# Autodesk Inventor assembly: Assembly
(part 3 of 3)
54. Universal_board_70x90mm_31x26-prt53
55. Universal_board_70x90mm_31x26-prt54
56. Universal_board_70x90mm_31x26-prt55
57. Universal_board_70x90mm_31x26-prt56
58. Universal_board_70x90mm_31x26-prt57
59. Universal_board_70x90mm_31x26-prt58
60. Universal_board_70x90mm_31x26-prt59
61. Universal_board_70x90mm_31x26-prt60
62. Universal_board_70x90mm_31x26-prt61
63. Universal_board_70x90mm_31x26-prt62
64. Universal_board_70x90mm_31x26-prt63
65. Universal_board_70x90mm_31x26-prt64
66. Universal_board_70x90mm_31x26-prt65
67. Universal_board_70x90mm_31x26-prt66
68. Universal_board_70x90mm_31x26-prt67
69. Universal_board_70x90mm_31x26-prt68
70. Universal_board_70x90mm_31x26-prt69
71. Universal_board_70x90mm_31x26-prt70
72. Universal_board_70x90mm_31x26-prt71
73. Universal_board_70x90mm_31x26-prt72
74. Universal_board_70x90mm_31x26-prt73
75. Universal_board_70x90mm_31x26-prt74
76. Universal_board_70x90mm_31x26-prt75
77. Universal_board_70x90mm_31x26-prt76
78. Universal_board_70x90mm_31x26-prt77
79. Universal_board_70x90mm_31x26-prt78
80. Universal_board_70x90mm_31x26-prt79
81. Universal_board_70x90mm_31x26-prt80
82. Universal_board_70x90mm_31x26-prt81
83. Universal_board_70x90mm_31x26-prt82
84. Universal_board_70x90mm_31x26-prt83
85. Universal_board_70x90mm_31x26-prt84
86. Universal_board_70x90mm_31x26-prt85
87. Universal_board_70x90mm_31x26-prt86
88. Universal_board_70x90mm_31x26-prt87
89. Universal_board_70x90mm_31x26-prt88
90. Universal_board_70x90mm_31x26-prt89
91. Universal_board_70x90mm_31x26-prt90
92. Universal_board_70x90mm_31x26-prt91
93. Universal_board_70x90mm_31x26-prt92
94. Universal_board_70x90mm_31x26-prt93
95. Universal_board_70x90mm_31x26-prt94
96. Universal_board_70x90mm_31x26-prt95
97. Universal_board_70x90mm_31x26-prt96
98. Universal_board_70x90mm_31x26-prt97
99. Universal_board_70x90mm_31x26-prt98
100. Universal_board_70x90mm_31x26-prt99
101. Universal_board_70x90mm_31x26-prt100
102. Universal_board_70x90mm_31x26-prt101
103. Universal_board_70x90mm_31x26-prt102
104. Universal_board_70x90mm_31x26-prt103
105. Universal_board_70x90mm_31x26-prt104
106. Universal_board_70x90mm_31x26-prt105
107. Universal_board_70x90mm_31x26-prt106
108. Universal_board_70x90mm_31x26-prt107
109. Universal_board_70x90mm_31x26-prt108
110. Universal_board_70x90mm_31x26-prt109
111. Universal_board_70x90mm_31x26-prt110
112. Universal_board_70x90mm_31x26-prt111
113. Universal_board_70x90mm_31x26-prt112
114. Universal_board_70x90mm_31x26-prt113
115. Universal_board_70x90mm_31x26-prt114
116. Universal_board_70x90mm_31x26-prt115
117. Universal_board_70x90mm_31x26-prt116
118. Universal_board_70x90mm_31x26-prt117
119. Universal_board_70x90mm_31x26-prt118
120. Universal_board_70x90mm_31x26-prt119
121. Universal_board_70x90mm_31x26-prt120
122. Universal_board_70x90mm_31x26-prt121
123. Universal_board_70x90mm_31x26-prt122
124. Universal_board_70x90mm_31x26-prt123
125. Universal_board_70x90mm_31x26-prt124
126. Universal_board_70x90mm_31x26-prt125
127. Universal_board_70x90mm_31x26-prt126
128. Universal_board_70x90mm_31x26-prt127
129. Universal_board_70x90mm_31x26-prt128
130. Universal_board_70x90mm_31x26-prt129
131. Universal_board_70x90mm_31x26-prt130
132. Universal_board_70x90mm_31x26-prt131
133. Universal_board_70x90mm_31x26-prt132
134. Universal_board_70x90mm_31x26-prt133
135. Universal_board_70x90mm_31x26-prt134
136. Universal_board_70x90mm_31x26-prt135
137. Universal_board_70x90mm_31x26-prt136
138. Universal_board_70x90mm_31x26-prt137
139. Universal_board_70x90mm_31x26-prt138
140. Universal_board_70x90mm_31x26-prt139
141. Universal_board_70x90mm_31x26-prt140
142. Universal_board_70x90mm_31x26-prt141
143. Universal_board_70x90mm_31x26-prt142
144. Universal_board_70x90mm_31x26-prt143
145. Universal_board_70x90mm_31x26-prt144
146. Universal_board_70x90mm_31x26-prt145
147. Universal_board_70x90mm_31x26-prt146
148. Universal_board_70x90mm_31x26-prt147
149. Universal_board_70x90mm_31x26-prt148
150. Universal_board_70x90mm_31x26-prt149
151. Universal_board_70x90mm_31x26-prt150
152. Universal_board_70x90mm_31x26-prt151
153. Universal_board_70x90mm_31x26-prt152
154. Universal_board_70x90mm_31x26-prt153
155. Universal_board_70x90mm_31x26-prt154
156. Universal_board_70x90mm_31x26-prt155
157. Universal_board_70x90mm_31x26-prt156
158. Universal_board_70x90mm_31x26-prt157
159. Universal_board_70x90mm_31x26-prt158
160. Universal_board_70x90mm_31x26-prt159
161. Universal_board_70x90mm_31x26-prt160
162. Universal_board_70x90mm_31x26-prt161
163. Universal_board_70x90mm_31x26-prt162
164. Universal_board_70x90mm_31x26-prt163
165. Universal_board_70x90mm_31x26-prt164
166. Universal_board_70x90mm_31x26-prt165
167. Universal_board_70x90mm_31x26-prt166
168. Universal_board_70x90mm_31x26-prt167
169. Universal_board_70x90mm_31x26-prt168
170. Universal_board_70x90mm_31x26-prt169
171. Universal_board_70x90mm_31x26-prt170
172. Universal_board_70x90mm_31x26-prt171
173. Universal_board_70x90mm_31x26-prt172
174. Universal_board_70x90mm_31x26-prt173
175. Universal_board_70x90mm_31x26-prt174
176. Universal_board_70x90mm_31x26-prt175
177. Universal_board_70x90mm_31x26-prt176
178. Universal_board_70x90mm_31x26-prt177
179. Universal_board_70x90mm_31x26-prt178
180. Universal_board_70x90mm_31x26-prt179
181. Universal_board_70x90mm_31x26-prt180
182. Universal_board_70x90mm_31x26-prt181
183. Universal_board_70x90mm_31x26-prt182
184. Universal_board_70x90mm_31x26-prt183
185. Universal_board_70x90mm_31x26-prt184
186. Universal_board_70x90mm_31x26-prt185
187. Universal_board_70x90mm_31x26-prt186
188. Universal_board_70x90mm_31x26-prt187
189. Universal_board_70x90mm_31x26-prt188
190. Universal_board_70x90mm_31x26-prt189
191. Universal_board_70x90mm_31x26-prt190
192. Universal_board_70x90mm_31x26-prt191
193. Universal_board_70x90mm_31x26-prt192
194. Universal_board_70x90mm_31x26-prt193
195. Universal_board_70x90mm_31x26-prt194
196. Universal_board_70x90mm_31x26-prt195
197. Universal_board_70x90mm_31x26-prt196
198. Universal_board_70x90mm_31x26-prt197
199. Universal_board_70x90mm_31x26-prt198
200. Universal_board_70x90mm_31x26-prt199
201. Universal_board_70x90mm_31x26-prt200
202. Universal_board_70x90mm_31x26-prt201
203. Universal_board_70x90mm_31x26-prt202
204. Universal_board_70x90mm_31x26-prt203
205. Universal_board_70x90mm_31x26-prt204
206. Universal_board_70x90mm_31x26-prt205
207. Universal_board_70x90mm_31x26-prt206
208. Universal_board_70x90mm_31x26-prt207
209. Universal_board_70x90mm_31x26-prt208
210. Universal_board_70x90mm_31x26-prt209
211. Universal_board_70x90mm_31x26-prt210
212. Universal_board_70x90mm_31x26-prt211
213. Universal_board_70x90mm_31x26-prt212
214. Universal_board_70x90mm_31x26-prt213
215. Universal_board_70x90mm_31x26-prt214
216. Universal_board_70x90mm_31x26-prt215
217. Universal_board_70x90mm_31x26-prt216
218. Universal_board_70x90mm_31x26-prt217
219. Universal_board_70x90mm_31x26-prt218
220. Universal_board_70x90mm_31x26-prt219
221. Universal_board_70x90mm_31x26-prt220
222. Universal_board_70x90mm_31x26-prt221
223. Universal_board_70x90mm_31x26-prt222
224. Universal_board_70x90mm_31x26-prt223
225. Universal_board_70x90mm_31x26-prt224
226. Universal_board_70x90mm_31x26-prt225
227. Universal_board_70x90mm_31x26-prt226
228. Universal_board_70x90mm_31x26-prt227
229. Universal_board_70x90mm_31x26-prt228
230. Universal_board_70x90mm_31x26-prt229
231. Universal_board_70x90mm_31x26-prt230
232. Universal_board_70x90mm_31x26-prt231
233. Universal_board_70x90mm_31x26-prt232
234. Universal_board_70x90mm_31x26-prt233
235. Universal_board_70x90mm_31x26-prt234
236. Universal_board_70x90mm_31x26-prt235
237. Universal_board_70x90mm_31x26-prt236
238. Universal_board_70x90mm_31x26-prt237
239. Universal_board_70x90mm_31x26-prt238
240. Universal_board_70x90mm_31x26-prt239
241. Universal_board_70x90mm_31x26-prt240
242. Universal_board_70x90mm_31x26-prt241
243. Universal_board_70x90mm_31x26-prt242
244. Universal_board_70x90mm_31x26-prt243
245. Universal_board_70x90mm_31x26-prt244
246. Universal_board_70x90mm_31x26-prt245
247. Universal_board_70x90mm_31x26-prt246
248. Universal_board_70x90mm_31x26-prt247
249. Universal_board_70x90mm_31x26-prt248
250. Universal_board_70x90mm_31x26-prt249
251. Universal_board_70x90mm_31x26-prt250
252. Universal_board_70x90mm_31x26-prt251
253. Universal_board_70x90mm_31x26-prt252
254. Universal_board_70x90mm_31x26-prt253
255. Universal_board_70x90mm_31x26-prt254
256. Universal_board_70x90mm_31x26-prt255
257. Universal_board_70x90mm_31x26-prt256
258. Universal_board_70x90mm_31x26-prt257
259. Universal_board_70x90mm_31x26-prt258
260. Universal_board_70x90mm_31x26-prt259
261. Universal_board_70x90mm_31x26-prt260
262. Universal_board_70x90mm_31x26-prt261
263. Universal_board_70x90mm_31x26-prt262
264. Universal_board_70x90mm_31x26-prt263
265. Universal_board_70x90mm_31x26-prt264
266. Universal_board_70x90mm_31x26-prt265
267. Universal_board_70x90mm_31x26-prt266
268. Universal_board_70x90mm_31x26-prt267
269. Universal_board_70x90mm_31x26-prt268
270. Universal_board_70x90mm_31x26-prt269
271. Universal_board_70x90mm_31x26-prt270
272. Universal_board_70x90mm_31x26-prt271
273. Universal_board_70x90mm_31x26-prt272
274. Universal_board_70x90mm_31x26-prt273
275. Universal_board_70x90mm_31x26-prt274
276. Universal_board_70x90mm_31x26-prt275
277. Universal_board_70x90mm_31x26-prt276
278. Universal_board_70x90mm_31x26-prt277
279. Universal_board_70x90mm_31x26-prt278
280. Universal_board_70x90mm_31x26-prt279
281. Universal_board_70x90mm_31x26-prt280
282. Universal_board_70x90mm_31x26-prt281
283. Universal_board_70x90mm_31x26-prt282
284. Universal_board_70x90mm_31x26-prt283
285. Universal_board_70x90mm_31x26-prt284
286. Universal_board_70x90mm_31x26-prt285
287. Universal_board_70x90mm_31x26-prt286
288. Universal_board_70x90mm_31x26-prt287
289. Universal_board_70x90mm_31x26-prt288
290. Universal_board_70x90mm_31x26-prt289
291. Universal_board_70x90mm_31x26-prt290
292. Universal_board_70x90mm_31x26-prt291
293. Universal_board_70x90mm_31x26-prt292
294. Universal_board_70x90mm_31x26-prt293
295. Universal_board_70x90mm_31x26-prt294
296. Universal_board_70x90mm_31x26-prt295
297. Universal_board_70x90mm_31x26-prt296
298. Universal_board_70x90mm_31x26-prt297
299. Universal_board_70x90mm_31x26-prt298
300. Universal_board_70x90mm_31x26-prt299
301. Universal_board_70x90mm_31x26-prt300
302. Universal_board_70x90mm_31x26-prt301
303. Universal_board_70x90mm_31x26-prt302
304. Universal_board_70x90mm_31x26-prt303
305. Universal_board_70x90mm_31x26-prt304
306. Universal_board_70x90mm_31x26-prt305
307. Universal_board_70x90mm_31x26-prt306
308. Universal_board_70x90mm_31x26-prt307
309. Universal_board_70x90mm_31x26-prt308
310. Universal_board_70x90mm_31x26-prt309
311. Universal_board_70x90mm_31x26-prt310
312. Universal_board_70x90mm_31x26-prt311
313. Universal_board_70x90mm_31x26-prt312
314. Universal_board_70x90mm_31x26-prt313
315. Universal_board_70x90mm_31x26-prt314
316. Universal_board_70x90mm_31x26-prt315
317. Universal_board_70x90mm_31x26-prt316
318. Universal_board_70x90mm_31x26-prt317
319. Universal_board_70x90mm_31x26-prt318
320. Universal_board_70x90mm_31x26-prt319
321. Universal_board_70x90mm_31x26-prt320
322. Universal_board_70x90mm_31x26-prt321
323. Universal_board_70x90mm_31x26-prt322
324. Universal_board_70x90mm_31x26-prt323
325. Universal_board_70x90mm_31x26-prt324
326. Universal_board_70x90mm_31x26-prt325
327. Universal_board_70x90mm_31x26-prt326
328. Universal_board_70x90mm_31x26-prt327
329. Universal_board_70x90mm_31x26-prt328
330. Universal_board_70x90mm_31x26-prt329
331. Universal_board_70x90mm_31x26-prt330
332. Universal_board_70x90mm_31x26-prt331
333. Universal_board_70x90mm_31x26-prt332
334. Universal_board_70x90mm_31x26-prt333
335. Universal_board_70x90mm_31x26-prt334
336. Universal_board_70x90mm_31x26-prt335
337. Universal_board_70x90mm_31x26-prt336
338. Universal_board_70x90mm_31x26-prt337
339. Universal_board_70x90mm_31x26-prt338
340. Universal_board_70x90mm_31x26-prt339
341. Universal_board_70x90mm_31x26-prt340
342. Universal_board_70x90mm_31x26-prt341
343. Universal_board_70x90mm_31x26-prt342
344. Universal_board_70x90mm_31x26-prt343
345. Universal_board_70x90mm_31x26-prt344
346. Universal_board_70x90mm_31x26-prt345
347. Universal_board_70x90mm_31x26-prt346
348. Universal_board_70x90mm_31x26-prt347
349. Universal_board_70x90mm_31x26-prt348
350. Universal_board_70x90mm_31x26-prt349
351. Universal_board_70x90mm_31x26-prt350
352. Universal_board_70x90mm_31x26-prt351
353. Universal_board_70x90mm_31x26-prt352
354. Universal_board_70x90mm_31x26-prt353
355. Universal_board_70x90mm_31x26-prt354
356. Universal_board_70x90mm_31x26-prt355
357. Universal_board_70x90mm_31x26-prt356
358. Universal_board_70x90mm_31x26-prt357
359. Universal_board_70x90mm_31x26-prt358
360. Universal_board_70x90mm_31x26-prt359
361. Universal_board_70x90mm_31x26-prt360
362. Universal_board_70x90mm_31x26-prt361
363. Universal_board_70x90mm_31x26-prt362
364. Universal_board_70x90mm_31x26-prt363
365. Universal_board_70x90mm_31x26-prt364
366. Universal_board_70x90mm_31x26-prt365
367. Universal_board_70x90mm_31x26-prt366
368. Universal_board_70x90mm_31x26-prt367
369. Universal_board_70x90mm_31x26-prt368
370. Universal_board_70x90mm_31x26-prt369
371. Universal_board_70x90mm_31x26-prt370
372. Universal_board_70x90mm_31x26-prt371
373. Universal_board_70x90mm_31x26-prt372
374. Universal_board_70x90mm_31x26-prt373
375. Universal_board_70x90mm_31x26-prt374
376. Universal_board_70x90mm_31x26-prt375
377. Universal_board_70x90mm_31x26-prt376
378. Universal_board_70x90mm_31x26-prt377
379. Universal_board_70x90mm_31x26-prt378
380. Universal_board_70x90mm_31x26-prt379
381. Universal_board_70x90mm_31x26-prt380
382. Universal_board_70x90mm_31x26-prt381
383. Universal_board_70x90mm_31x26-prt382
384. Universal_board_70x90mm_31x26-prt383
385. Universal_board_70x90mm_31x26-prt384
386. Universal_board_70x90mm_31x26-prt385
387. Universal_board_70x90mm_31x26-prt386
388. Universal_board_70x90mm_31x26-prt387
389. Universal_board_70x90mm_31x26-prt388
390. Universal_board_70x90mm_31x26-prt389
391. Universal_board_70x90mm_31x26-prt390
392. Universal_board_70x90mm_31x26-prt391
393. Universal_board_70x90mm_31x26-prt392
394. Universal_board_70x90mm_31x26-prt393
395. Universal_board_70x90mm_31x26-prt394
396. Universal_board_70x90mm_31x26-prt395
397. Universal_board_70x90mm_31x26-prt396
398. Universal_board_70x90mm_31x26-prt397
399. Universal_board_70x90mm_31x26-prt398
400. Universal_board_70x90mm_31x26-prt399
401. Universal_board_70x90mm_31x26-prt400
402. Universal_board_70x90mm_31x26-prt401
403. Universal_board_70x90mm_31x26-prt402
404. Universal_board_70x90mm_31x26-prt403
405. Universal_board_70x90mm_31x26-prt404
406. Universal_board_70x90mm_31x26-prt405
407. Universal_board_70x90mm_31x26-prt406
408. Universal_board_70x90mm_31x26-prt407
409. Universal_board_70x90mm_31x26-prt408
410. Universal_board_70x90mm_31x26-prt409
411. Universal_board_70x90mm_31x26-prt410
412. Universal_board_70x90mm_31x26-prt411
413. Universal_board_70x90mm_31x26-prt412
414. Universal_board_70x90mm_31x26-prt413
415. Universal_board_70x90mm_31x26-prt414
416. Universal_board_70x90mm_31x26-prt415
417. Universal_board_70x90mm_31x26-prt416
418. Universal_board_70x90mm_31x26-prt417
419. Universal_board_70x90mm_31x26-prt418
420. Universal_board_70x90mm_31x26-prt419
421. Universal_board_70x90mm_31x26-prt420
422. Universal_board_70x90mm_31x26-prt421
423. Universal_board_70x90mm_31x26-prt422
424. Universal_board_70x90mm_31x26-prt423
425. Universal_board_70x90mm_31x26-prt424
426. Universal_board_70x90mm_31x26-prt425
427. Universal_board_70x90mm_31x26-prt426
428. Universal_board_70x90mm_31x26-prt427
429. Universal_board_70x90mm_31x26-prt428
430. Universal_board_70x90mm_31x26-prt429
431. Universal_board_70x90mm_31x26-prt430
432. Universal_board_70x90mm_31x26-prt431
433. Universal_board_70x90mm_31x26-prt432
434. Universal_board_70x90mm_31x26-prt433
435. Universal_board_70x90mm_31x26-prt434
436. Universal_board_70x90mm_31x26-prt435
437. Universal_board_70x90mm_31x26-prt436
438. Universal_board_70x90mm_31x26-prt437
439. Universal_board_70x90mm_31x26-prt438
440. Universal_board_70x90mm_31x26-prt439
441. Universal_board_70x90mm_31x26-prt440
442. Universal_board_70x90mm_31x26-prt441
443. Universal_board_70x90mm_31x26-prt442
444. Universal_board_70x90mm_31x26-prt443
445. Universal_board_70x90mm_31x26-prt444
446. Universal_board_70x90mm_31x26-prt445
447. Universal_board_70x90mm_31x26-prt446
448. Universal_board_70x90mm_31x26-prt447
449. Universal_board_70x90mm_31x26-prt448
450. Universal_board_70x90mm_31x26-prt449
451. Universal_board_70x90mm_31x26-prt450
452. Universal_board_70x90mm_31x26-prt451
453. Universal_board_70x90mm_31x26-prt452
454. Universal_board_70x90mm_31x26-prt453
455. Universal_board_70x90mm_31x26-prt454
456. Universal_board_70x90mm_31x26-prt455
457. Universal_board_70x90mm_31x26-prt456
458. Universal_board_70x90mm_31x26-prt457
459. Universal_board_70x90mm_31x26-prt458
460. Universal_board_70x90mm_31x26-prt459
461. Universal_board_70x90mm_31x26-prt460
462. Universal_board_70x90mm_31x26-prt461
463. Universal_board_70x90mm_31x26-prt462
464. Universal_board_70x90mm_31x26-prt463
465. Universal_board_70x90mm_31x26-prt464
466. Universal_board_70x90mm_31x26-prt465
467. Universal_board_70x90mm_31x26-prt466
468. Universal_board_70x90mm_31x26-prt467
469. Universal_board_70x90mm_31x26-prt468
470. Universal_board_70x90mm_31x26-prt469
471. Universal_board_70x90mm_31x26-prt470
472. Universal_board_70x90mm_31x26-prt471
473. Universal_board_70x90mm_31x26-prt472
474. Universal_board_70x90mm_31x26-prt473
475. Universal_board_70x90mm_31x26-prt474
476. Universal_board_70x90mm_31x26-prt475
477. Universal_board_70x90mm_31x26-prt476
478. Universal_board_70x90mm_31x26-prt477
479. Universal_board_70x90mm_31x26-prt478
480. Universal_board_70x90mm_31x26-prt479
481. Universal_board_70x90mm_31x26-prt480
482. Universal_board_70x90mm_31x26-prt481
483. Universal_board_70x90mm_31x26-prt482
484. Universal_board_70x90mm_31x26-prt483
485. Universal_board_70x90mm_31x26-prt484
486. Universal_board_70x90mm_31x26-prt485
487. Universal_board_70x90mm_31x26-prt486
488. Universal_board_70x90mm_31x26-prt487
489. Universal_board_70x90mm_31x26-prt488
490. Universal_board_70x90mm_31x26-prt489
491. Universal_board_70x90mm_31x26-prt490
492. Universal_board_70x90mm_31x26-prt491
493. Universal_board_70x90mm_31x26-prt492
494. Universal_board_70x90mm_31x26-prt493
495. Universal_board_70x90mm_31x26-prt494
496. Universal_board_70x90mm_31x26-prt495
497. Universal_board_70x90mm_31x26-prt496
498. Universal_board_70x90mm_31x26-prt497
499. Universal_board_70x90mm_31x26-prt498
500. Universal_board_70x90mm_31x26-prt499
501. Universal_board_70x90mm_31x26-prt500
502. Universal_board_70x90mm_31x26-prt501
503. Universal_board_70x90mm_31x26-prt502
504. Universal_board_70x90mm_31x26-prt503
505. Universal_board_70x90mm_31x26-prt504
506. Universal_board_70x90mm_31x26-prt505
507. Universal_board_70x90mm_31x26-prt506
508. Universal_board_70x90mm_31x26-prt507
509. Universal_board_70x90mm_31x26-prt508
510. Universal_board_70x90mm_31x26-prt509
511. Universal_board_70x90mm_31x26-prt510
512. Universal_board_70x90mm_31x26-prt511
513. Universal_board_70x90mm_31x26-prt512
514. Universal_board_70x90mm_31x26-prt513
515. Universal_board_70x90mm_31x26-prt514
516. Universal_board_70x90mm_31x26-prt515
517. Universal_board_70x90mm_31x26-prt516
518. Universal_board_70x90mm_31x26-prt517
519. Universal_board_70x90mm_31x26-prt518
520. Universal_board_70x90mm_31x26-prt519
521. Universal_board_70x90mm_31x26-prt520
522. Universal_board_70x90mm_31x26-prt521
523. Universal_board_70x90mm_31x26-prt522
524. Universal_board_70x90mm_31x26-prt523
525. Universal_board_70x90mm_31x26-prt524
526. Universal_board_70x90mm_31x26-prt525
527. Universal_board_70x90mm_31x26-prt526
528. Universal_board_70x90mm_31x26-prt527
529. Universal_board_70x90mm_31x26-prt528
530. Universal_board_70x90mm_31x26-prt529
531. Universal_board_70x90mm_31x26-prt530
532. Universal_board_70x90mm_31x26-prt531
533. Universal_board_70x90mm_31x26-prt532
534. Universal_board_70x90mm_31x26-prt533
535. Universal_board_70x90mm_31x26-prt534
536. Universal_board_70x90mm_31x26-prt535
537. Universal_board_70x90mm_31x26-prt536
538. Universal_board_70x90mm_31x26-prt537
539. Universal_board_70x90mm_31x26-prt538
540. Universal_board_70x90mm_31x26-prt539
541. Universal_board_70x90mm_31x26-prt540
542. Universal_board_70x90mm_31x26-prt541
543. Universal_board_70x90mm_31x26-prt542
544. Universal_board_70x90mm_31x26-prt543
545. Universal_board_70x90mm_31x26-prt544
546. Universal_board_70x90mm_31x26-prt545
547. Universal_board_70x90mm_31x26-prt546
548. Universal_board_70x90mm_31x26-prt547
549. Universal_board_70x90mm_31x26-prt548
550. Universal_board_70x90mm_31x26-prt549
551. Universal_board_70x90mm_31x26-prt550
552. Universal_board_70x90mm_31x26-prt551
553. Universal_board_70x90mm_31x26-prt552
554. Universal_board_70x90mm_31x26-prt553
555. Universal_board_70x90mm_31x26-prt554
556. Universal_board_70x90mm_31x26-prt555
557. Universal_board_70x90mm_31x26-prt556
558. Universal_board_70x90mm_31x26-prt557
559. Universal_board_70x90mm_31x26-prt558
560. Universal_board_70x90mm_31x26-prt559
561. Universal_board_70x90mm_31x26-prt560
562. Universal_board_70x90mm_31x26-prt561
563. Universal_board_70x90mm_31x26-prt562
564. Universal_board_70x90mm_31x26-prt563
565. Universal_board_70x90mm_31x26-prt564
566. Universal_board_70x90mm_31x26-prt565
567. Universal_board_70x90mm_31x26-prt566
568. Universal_board_70x90mm_31x26-prt567
569. Universal_board_70x90mm_31x26-prt568
570. Universal_board_70x90mm_31x26-prt569
571. Universal_board_70x90mm_31x26-prt570
572. Universal_board_70x90mm_31x26-prt571
573. Universal_board_70x90mm_31x26-prt572
574. Universal_board_70x90mm_31x26-prt573
575. Universal_board_70x90mm_31x26-prt574
576. Universal_board_70x90mm_31x26-prt575
577. Universal_board_70x90mm_31x26-prt576
578. Universal_board_70x90mm_31x26-prt577
579. Universal_board_70x90mm_31x26-prt578
580. Universal_board_70x90mm_31x26-prt579
581. Universal_board_70x90mm_31x26-prt580
582. Universal_board_70x90mm_31x26-prt581
583. Universal_board_70x90mm_31x26-prt582
584. Universal_board_70x90mm_31x26-prt583
585. Universal_board_70x90mm_31x26-prt584
586. Universal_board_70x90mm_31x26-prt585
587. Universal_board_70x90mm_31x26-prt586
588. Universal_board_70x90mm_31x26-prt587
589. Universal_board_70x90mm_31x26-prt588
590. Universal_board_70x90mm_31x26-prt589
591. Universal_board_70x90mm_31x26-prt590
592. Universal_board_70x90mm_31x26-prt591
593. Universal_board_70x90mm_31x26-prt592
594. Universal_board_70x90mm_31x26-prt593
595. Universal_board_70x90mm_31x26-prt594
596. Universal_board_70x90mm_31x26-prt595
597. Universal_board_70x90mm_31x26-prt596
598. Universal_board_70x90mm_31x26-prt597
599. Universal_board_70x90mm_31x26-prt598
600. Universal_board_70x90mm_31x26-prt599
601. Universal_board_70x90mm_31x26-prt600
602. Universal_board_70x90mm_31x26-prt601
603. Universal_board_70x90mm_31x26-prt602
604. Universal_board_70x90mm_31x26-prt603
605. Universal_board_70x90mm_31x26-prt604
606. Universal_board_70x90mm_31x26-prt605
607. Universal_board_70x90mm_31x26-prt606
608. Universal_board_70x90mm_31x26-prt607
609. Universal_board_70x90mm_31x26-prt608
610. Universal_board_70x90mm_31x26-prt609
611. Universal_board_70x90mm_31x26-prt610
612. Universal_board_70x90mm_31x26-prt611
613. Universal_board_70x90mm_31x26-prt612
614. Universal_board_70x90mm_31x26-prt613
615. Universal_board_70x90mm_31x26-prt614
616. Universal_board_70x90mm_31x26-prt615
617. Universal_board_70x90mm_31x26-prt616
618. Universal_board_70x90mm_31x26-prt617
619. Universal_board_70x90mm_31x26-prt618
620. Universal_board_70x90mm_31x26-prt619
621. Universal_board_70x90mm_31x26-prt620
622. Universal_board_70x90mm_31x26-prt621
623. Universal_board_70x90mm_31x26-prt622
624. Universal_board_70x90mm_31x26-prt623
625. Universal_board_70x90mm_31x26-prt624
626. Universal_board_70x90mm_31x26-prt625
627. Universal_board_70x90mm_31x26-prt626
628. Universal_board_70x90mm_31x26-prt627
629. Universal_board_70x90mm_31x26-prt628
630. Universal_board_70x90mm_31x26-prt629
631. Universal_board_70x90mm_31x26-prt630
632. Universal_board_70x90mm_31x26-prt631
633. Universal_board_70x90mm_31x26-prt632
634. Universal_board_70x90mm_31x26-prt633
635. Universal_board_70x90mm_31x26-prt634
636. Universal_board_70x90mm_31x26-prt635
637. Universal_board_70x90mm_31x26-prt636
638. Universal_board_70x90mm_31x26-prt637
639. Universal_board_70x90mm_31x26-prt638
640. Universal_board_70x90mm_31x26-prt639
641. Universal_board_70x90mm_31x26-prt640
642. Universal_board_70x90mm_31x26-prt641
643. Universal_board_70x90mm_31x26-prt642
644. Universal_board_70x90mm_31x26-prt643
645. Universal_board_70x90mm_31x26-prt644
646. Universal_board_70x90mm_31x26-prt645
647. Universal_board_70x90mm_31x26-prt646
648. Universal_board_70x90mm_31x26-prt647
649. Universal_board_70x90mm_31x26-prt648
650. Universal_board_70x90mm_31x26-prt649
651. Universal_board_70x90mm_31x26-prt650
652. Universal_board_70x90mm_31x26-prt651
653. Universal_board_70x90mm_31x26-prt652
654. Universal_board_70x90mm_31x26-prt653
655. Universal_board_70x90mm_31x26-prt654
656. Universal_board_70x90mm_31x26-prt655
657. Universal_board_70x90mm_31x26-prt656
658. Universal_board_70x90mm_31x26-prt657
659. Universal_board_70x90mm_31x26-prt658
660. Universal_board_70x90mm_31x26-prt659
661. Universal_board_70x90mm_31x26-prt660
662. Universal_board_70x90mm_31x26-prt661
663. Universal_board_70x90mm_31x26-prt662
664. Universal_board_70x90mm_31x26-prt663
665. Universal_board_70x90mm_31x26-prt664
666. Universal_board_70x90mm_31x26-prt665
667. Universal_board_70x90mm_31x26-prt666
668. Universal_board_70x90mm_31x26-prt667
669. Universal_board_70x90mm_31x26-prt668
670. Universal_board_70x90mm_31x26-prt669
671. Universal_board_70x90mm_31x26-prt670
672. Universal_board_70x90mm_31x26-prt671
673. Universal_board_70x90mm_31x26-prt672
674. Universal_board_70x90mm_31x26-prt673
675. Universal_board_70x90mm_31x26-prt674
676. Universal_board_70x90mm_31x26-prt675
677. Universal_board_70x90mm_31x26-prt676
678. Universal_board_70x90mm_31x26-prt677
679. Universal_board_70x90mm_31x26-prt678
680. Universal_board_70x90mm_31x26-prt679
681. Universal_board_70x90mm_31x26-prt680
682. Universal_board_70x90mm_31x26-prt681
683. Universal_board_70x90mm_31x26-prt682
684. Universal_board_70x90mm_31x26-prt683
685. Universal_board_70x90mm_31x26-prt684
686. Universal_board_70x90mm_31x26-prt685
687. Universal_board_70x90mm_31x26-prt686
688. Universal_board_70x90mm_31x26-prt687
689. Universal_board_70x90mm_31x26-prt688
690. Universal_board_70x90mm_31x26-prt689
691. Universal_board_70x90mm_31x26-prt690
692. Universal_board_70x90mm_31x26-prt691
693. Universal_board_70x90mm_31x26-prt692
694. Universal_board_70x90mm_31x26-prt693
695. Universal_board_70x90mm_31x26-prt694
696. Universal_board_70x90mm_31x26-prt695
697. Universal_board_70x90mm_31x26-prt696
698. Universal_board_70x90mm_31x26-prt697
699. Universal_board_70x90mm_31x26-prt698
700. Universal_board_70x90mm_31x26-prt699
701. Universal_board_70x90mm_31x26-prt700
702. Universal_board_70x90mm_31x26-prt701
703. Universal_board_70x90mm_31x26-prt702
704. Universal_board_70x90mm_31x26-prt703
705. Universal_board_70x90mm_31x26-prt704
706. Universal_board_70x90mm_31x26-prt705
707. Universal_board_70x90mm_31x26-prt706
708. Universal_board_70x90mm_31x26-prt707
709. Universal_board_70x90mm_31x26-prt708
710. Universal_board_70x90mm_31x26-prt709
711. Universal_board_70x90mm_31x26-prt710
712. Universal_board_70x90mm_31x26-prt711
713. Universal_board_70x90mm_31x26-prt712
714. Universal_board_70x90mm_31x26-prt713
715. Universal_board_70x90mm_31x26-prt714
716. Universal_board_70x90mm_31x26-prt715
717. Universal_board_70x90mm_31x26-prt716
718. Universal_board_70x90mm_31x26-prt717
719. Universal_board_70x90mm_31x26-prt718
720. Universal_board_70x90mm_31x26-prt719
721. Universal_board_70x90mm_31x26-prt720
722. Universal_board_70x90mm_31x26-prt721
723. Universal_board_70x90mm_31x26-prt722
724. Universal_board_70x90mm_31x26-prt723
725. Universal_board_70x90mm_31x26-prt724
726. Universal_board_70x90mm_31x26-prt725
727. Universal_board_70x90mm_31x26-prt726
728. Universal_board_70x90mm_31x26-prt727
729. Universal_board_70x90mm_31x26-prt728
730. Universal_board_70x90mm_31x26-prt729
731. Universal_board_70x90mm_31x26-prt730
732. Universal_board_70x90mm_31x26-prt731
733. Universal_board_70x90mm_31x26-prt732
734. Universal_board_70x90mm_31x26-prt733
735. Universal_board_70x90mm_31x26-prt734
736. Universal_board_70x90mm_31x26-prt735
737. Universal_board_70x90mm_31x26-prt736
738. Universal_board_70x90mm_31x26-prt737
739. Universal_board_70x90mm_31x26-prt738
740. Universal_board_70x90mm_31x26-prt739
741. Universal_board_70x90mm_31x26-prt740
742. Universal_board_70x90mm_31x26-prt741
743. Universal_board_70x90mm_31x26-prt742
744. Universal_board_70x90mm_31x26-prt743
745. Universal_board_70x90mm_31x26-prt744
746. Universal_board_70x90mm_31x26-prt745
747. Universal_board_70x90mm_31x26-prt746
748. Universal_board_70x90mm_31x26-prt747
749. Universal_board_70x90mm_31x26-prt748
750. Universal_board_70x90mm_31x26-prt749
751. Universal_board_70x90mm_31x26-prt750
752. Universal_board_70x90mm_31x26-prt751
753. Universal_board_70x90mm_31x26-prt752
754. Universal_board_70x90mm_31x26-prt753
755. Universal_board_70x90mm_31x26-prt754
756. Universal_board_70x90mm_31x26-prt755
757. Universal_board_70x90mm_31x26-prt756
758. Universal_board_70x90mm_31x26-prt757
759. Universal_board_70x90mm_31x26-prt758
760. Universal_board_70x90mm_31x26-prt759
761. Universal_board_70x90mm_31x26-prt760
762. Universal_board_70x90mm_31x26-prt761
763. Universal_board_70x90mm_31x26-prt762
764. Universal_board_70x90mm_31x26-prt763
765. Universal_board_70x90mm_31x26-prt764
766. Universal_board_70x90mm_31x26-prt765
767. Universal_board_70x90mm_31x26-prt766
768. Universal_board_70x90mm_31x26-prt767
769. Universal_board_70x90mm_31x26-prt768
770. Universal_board_70x90mm_31x26-prt769
771. Universal_board_70x90mm_31x26-prt770
772. Universal_board_70x90mm_31x26-prt771
773. Universal_board_70x90mm_31x26-prt772
774. Universal_board_70x90mm_31x26-prt773
775. Universal_board_70x90mm_31x26-prt774
776. Universal_board_70x90mm_31x26-prt775
777. Universal_board_70x90mm_31x26-prt776
778. Universal_board_70x90mm_31x26-prt777
779. Universal_board_70x90mm_31x26-prt778
780. Universal_board_70x90mm_31x26-prt779
781. Universal_board_70x90mm_31x26-prt780
782. Universal_board_70x90mm_31x26-prt781
783. Universal_board_70x90mm_31x26-prt782
784. Universal_board_70x90mm_31x26-prt783
785. Universal_board_70x90mm_31x26-prt784
786. Universal_board_70x90mm_31x26-prt785
787. Universal_board_70x90mm_31x26-prt786
788. Universal_board_70x90mm_31x26-prt787
789. Universal_board_70x90mm_31x26-prt788
790. Universal_board_70x90mm_31x26-prt789
791. Universal_board_70x90mm_31x26-prt790
792. Universal_board_70x90mm_31x26-prt791
793. Universal_board_70x90mm_31x26-prt792
794. Universal_board_70x90mm_31x26-prt793
795. Universal_board_70x90mm_31x26-prt794
796. Universal_board_70x90mm_31x26-prt795
797. Universal_board_70x90mm_31x26-prt796
798. Universal_board_70x90mm_31x26-prt797
799. Universal_board_70x90mm_31x26-prt798
800. Universal_board_70x90mm_31x26-prt799
801. Universal_board_70x90mm_31x26-prt800
802. Universal_board_70x90mm_31x26-prt801
803. Universal_board_70x90mm_31x26-prt802
804. Universal_board_70x90mm_31x26-prt803
805. Universal_board_70x90mm_31x26-prt804
806. Universal_board_70x90mm_31x26-prt805
807. Universal_board_70x90mm_31x26-prt806
808. Universal_board_70x90mm_31x26-prt807
809. Universal_board_70x90mm_31x26-prt808
810. Universal_board_70x90mm_31x26-prt809
811. Universal_board_70x90mm_31x26-prt810
812. Universal_board_70x90mm_31x26-prt811
813. Universal_board_70x90mm_31x26-prt812
814. Universal_board_70x90mm_31x26-prt813
815. Universal_board_70x90mm_31x26-prt814
816. Universal_board_70x90mm_31x26-prt815
817. Universal_board_70x90mm_31x26-prt816
818. Universal_board_70x90mm_31x26-prt817
819. Universal_board_70x90mm_31x26-prt818
820. Universal_board_70x90mm_31x26-prt819
821. Universal_board_70x90mm_31x26-prt820
822. Universal_board_70x90mm_31x26-prt821
823. Universal_board_70x90mm_31x26-prt822
824. Universal_board_70x90mm_31x26-prt823
825. Universal_board_70x90mm_31x26-prt824
826. Universal_board_70x90mm_31x26-prt825
827. Universal_board_70x90mm_31x26-prt826
828. Universal_board_70x90mm_31x26-prt827
829. Universal_board_70x90mm_31x26-prt828
830. Universal_board_70x90mm_31x26-prt829
831. Universal_board_70x90mm_31x26-prt830
832. Universal_board_70x90mm_31x26-prt831
833. Universal_board_70x90mm_31x26-prt832
834. Universal_board_70x90mm_31x26-prt833
835. Universal_board_70x90mm_31x26-prt834
836. Universal_board_70x90mm_31x26-prt835
837. Universal_board_70x90mm_31x26-prt836
838. Universal_board_70x90mm_31x26-prt837
839. Universal_board_70x90mm_31x26-prt838
840. Universal_board_70x90mm_31x26-prt839
841. Universal_board_70x90mm_31x26-prt840
842. Universal_board_70x90mm_31x26-prt841
843. Universal_board_70x90mm_31x26-prt842
844. Universal_board_70x90mm_31x26-prt843
845. Universal_board_70x90mm_31x26-prt844
846. Universal_board_70x90mm_31x26-prt845
847. Universal_board_70x90mm_31x26-prt846
848. Universal_board_70x90mm_31x26-prt847
849. Universal_board_70x90mm_31x26-prt848
850. Universal_board_70x90mm_31x26-prt849
851. Universal_board_70x90mm_31x26-prt850
852. Universal_board_70x90mm_31x26-prt851
853. Universal_board_70x90mm_31x26-prt852
854. Universal_board_70x90mm_31x26-prt853
855. Universal_board_70x90mm_31x26-prt854
856. Universal_board_70x90mm_31x26-prt855
857. Universal_board_70x90mm_31x26-prt856
858. Universal_board_70x90mm_31x26-prt857
859. Universal_board_70x90mm_31x26-prt858
860. Universal_board_70x90mm_31x26-prt859
861. Universal_board_70x90mm_31x26-prt860
862. Universal_board_70x90mm_31x26-prt861
863. Universal_board_70x90mm_31x26-prt862
864. Universal_board_70x90mm_31x26-prt863
865. Universal_board_70x90mm_31x26-prt864
866. Universal_board_70x90mm_31x26-prt865
867. Universal_board_70x90mm_31x26-prt866
868. Universal_board_70x90mm_31x26-prt867
869. Universal_board_70x90mm_31x26-prt868
870. Universal_board_70x90mm_31x26-prt869
871. Universal_board_70x90mm_31x26-prt870
872. Universal_board_70x90mm_31x26-prt871
873. Universal_board_70x90mm_31x26-prt872
874. Universal_board_70x90mm_31x26-prt873
875. Universal_board_70x90mm_31x26-prt874
876. Universal_board_70x90mm_31x26-prt875
877. Universal_board_70x90mm_31x26-prt876
878. Universal_board_70x90mm_31x26-prt877
879. Universal_board_70x90mm_31x26-prt878
880. Universal_board_70x90mm_31x26-prt879
881. Universal_board_70x90mm_31x26-prt880
882. Universal_board_70x90mm_31x26-prt881
883. Universal_board_70x90mm_31x26-prt882
884. Universal_board_70x90mm_31x26-prt883
885. Universal_board_70x90mm_31x26-prt884
886. Universal_board_70x90mm_31x26-prt885
887. Universal_board_70x90mm_31x26-prt886
888. Universal_board_70x90mm_31x26-prt887
889. Universal_board_70x90mm_31x26-prt888
890. Universal_board_70x90mm_31x26-prt889
891. Universal_board_70x90mm_31x26-prt890
892. Universal_board_70x90mm_31x26-prt891
893. Universal_board_70x90mm_31x26-prt892
894. Universal_board_70x90mm_31x26-prt893
895. Universal_board_70x90mm_31x26-prt894
896. Universal_board_70x90mm_31x26-prt895
897. Universal_board_70x90mm_31x26-prt896
898. Universal_board_70x90mm_31x26-prt897
899. Universal_board_70x90mm_31x26-prt898
900. Universal_board_70x90mm_31x26-prt899
901. Universal_board_70x90mm_31x26-prt900
902. Universal_board_70x90mm_31x26-prt901
903. Universal_board_70x90mm_31x26-prt902
904. Universal_board_70x90mm_31x26-prt903
905. Universal_board_70x90mm_31x26-prt904
906. Universal_board_70x90mm_31x26-prt905
907. Universal_board_70x90mm_31x26-prt906
